# Autodesk Inventor assembly: Babka
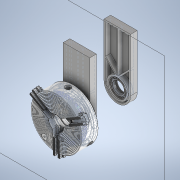
[picture p0: Inventor's stored thumbnail of the model, 180x180]
Saved by Autodesk Inventor 2022 (Build 260153000, 153)
## iProperties
Created: 2023-08-16
Part Number: Babka
Document SubType Name: Assembly
Designer: Kippi
Author: Kippi
## Documents named in this file (5)
- C:\Users\Kippi\Documents\CNC_Lathe\Babka.iam
- C:\Users\Kippi\Documents\CNC_Lathe\FlanecPodsipnikForwardBabka.ipt
- C:\Users\Kippi\Documents\Inventor\Content Center Files\R2022\en-US\GB_T 276-94 60000-2RS and 2LS\Bearing 6014-2RS GB_T 276-94.ipt
- C:\Users\Kippi\Documents\CNC_Lathe\Rails\3 JAW CHUCK SCROLL SLIDES REAR PLATE.ipt
- C:\Users\Kippi\Documents\CNC_Lathe\ShaibaNaPatron.ipt
## Components (6 placed, 4 different names)
1. FlanecPodsipnikForwardBabka:1 — Mate:1, Mate:2, Flush:3, Flush:4
2. Rolling bearing GB/T 276-1994 Type 60000-2RS and 2LS 6014-2RS:1 — Mate:1, Mate:2, Mate:5
3. Rolling bearing GB/T 276-1994 Type 60000-2RS and 2LS 6014-2RS:2 — Mate:6
4. 3 JAW CHUCK SCROLL SLIDES REAR PLATE:1 — Mate:3, Mate:4
5. ShaibaNaPatron:1 — Mate:3, Mate:4, Mate:5, Mate:6
6. FlanecPodsipnikForwardBabka:3 — Flush:3, Flush:4
## Relationships (8: Mate 6, Flush 2)
- Mate:1: FlanecPodsipnikForwardBabka:1 ↔ Rolling bearing GB/T 276-1994 Type 60000-2RS and 2LS 6014-2RS:1
- Mate:2: FlanecPodsipnikForwardBabka:1 ↔ Rolling bearing GB/T 276-1994 Type 60000-2RS and 2LS 6014-2RS:1
- Mate:3: 3 JAW CHUCK SCROLL SLIDES REAR PLATE:1 ↔ ShaibaNaPatron:1
- Mate:4: 3 JAW CHUCK SCROLL SLIDES REAR PLATE:1 ↔ ShaibaNaPatron:1
- Mate:5: Rolling bearing GB/T 276-1994 Type 60000-2RS and 2LS 6014-2RS:1 ↔ ShaibaNaPatron:1
- Mate:6: Rolling bearing GB/T 276-1994 Type 60000-2RS and 2LS 6014-2RS:2 ↔ ShaibaNaPatron:1
- Flush:3: FlanecPodsipnikForwardBabka:1 ↔ FlanecPodsipnikForwardBabka:3
- Flush:4: FlanecPodsipnikForwardBabka:1 ↔ FlanecPodsipnikForwardBabka:3
